# Autodesk Inventor assembly: port_starboard_side
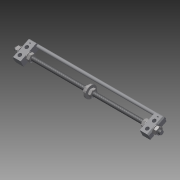
[picture p0: Inventor's stored thumbnail of the model, 180x180]
Saved by Autodesk Inventor 2015 (Build 190159000, 159)
## iProperties
Created: 2015-04-28
Part Number: port_starboard_side
Document SubType Name: Assembly
Designer: X
Author: X
## Documents named in this file (7)
- G:\3d printer\Prusa i3\CAD\port_starboard_side.iam
- G:\3d printer\Prusa i3\CAD\rod\M10-380-thread.ipt
- G:\3d printer\Prusa i3\CAD\3d_printer_part\y-corners.ipt
- G:\3d printer\Prusa i3\CAD\rod\M8-350-smooth.ipt
- D:\Inventor\Content Center Files\R2015\en-US\DIN 934\DIN 934 - M10 x 1.25.ipt
- D:\Inventor\Content Center Files\R2015\en-US\ISO 7089\ISO 7089 - 10 - 140 HV(1).ipt
- D:\Inventor\Content Center Files\R2015\en-US\ISO 7093 A\ISO 7093 A - ST 10 - 140 HV .ipt
## Components (16 placed, 6 different names)
1. M10-380-thread:1 — Cylindrical:1, Cylindrical:2, Cylindrical:3, Cylindrical:4, Cylindrical:5, Cylindrical:6, Cylindrical:7, Cylindrical:8
2. y-corners:1 — Insert:2, Cylindrical:2, Insert:5, Insert:9
3. y-corners:2 — Insert:3, Cylindrical:1, Insert:4, Insert:8
4. M8-350-smooth:1 — Insert:2, Insert:3
5. ISO 7089 10 - 140 HV:2 — Insert:5, Insert:7
6. ISO 7089 10 - 140 HV:1 — Insert:4, Insert:6
7. DIN 934 - replaced by DIN EN 24032/28673/28674 M10 x 1.25:1 — Insert:7
8. DIN 934 - replaced by DIN EN 24032/28673/28674 M10 x 1.25:2 — Insert:6
9. ISO 7089 10 - 140 HV:3 — Insert:8, Mate:1
10. ISO 7089 10 - 140 HV:4 — Insert:9, Mate:2
11. DIN 934 - replaced by DIN EN 24032/28673/28674 M10 x 1.25:3 — Cylindrical:3, Mate:1
12. DIN 934 - replaced by DIN EN 24032/28673/28674 M10 x 1.25:4 — Cylindrical:4, Mate:2
13. ISO 7093 A ST 10 - 140 HV - A:1 — Cylindrical:5, Mate:3, Mate:4
14. ISO 7093 A ST 10 - 140 HV - A:2 — Cylindrical:6, Mate:3, Mate:5
15. DIN 934 - replaced by DIN EN 24032/28673/28674 M10 x 1.25:5 — Cylindrical:8, Mate:4
16. DIN 934 - replaced by DIN EN 24032/28673/28674 M10 x 1.25:6 — Cylindrical:7, Mate:5
## Relationships (21: Insert 8, CylindricalJoint 8, Mate 5)
- Insert:2: y-corners:1 ↔ M8-350-smooth:1
- Insert:3: y-corners:2 ↔ M8-350-smooth:1
- Cylindrical:1: M10-380-thread:1 ↔ y-corners:2
- Cylindrical:2: M10-380-thread:1 ↔ y-corners:1
- Insert:4: y-corners:2 ↔ ISO 7089 10 - 140 HV:1
- Insert:5: y-corners:1 ↔ ISO 7089 10 - 140 HV:2
- Insert:6: ISO 7089 10 - 140 HV:1 ↔ DIN 934 - replaced by DIN EN 24032/28673/28674 M10 x 1.25:2
- Insert:7: ISO 7089 10 - 140 HV:2 ↔ DIN 934 - replaced by DIN EN 24032/28673/28674 M10 x 1.25:1
- Insert:8: y-corners:2 ↔ ISO 7089 10 - 140 HV:3
- Insert:9: y-corners:1 ↔ ISO 7089 10 - 140 HV:4
- Cylindrical:3: M10-380-thread:1 ↔ DIN 934 - replaced by DIN EN 24032/28673/28674 M10 x 1.25:3
- Mate:1: ISO 7089 10 - 140 HV:3 ↔ DIN 934 - replaced by DIN EN 24032/28673/28674 M10 x 1.25:3
- Cylindrical:4: M10-380-thread:1 ↔ DIN 934 - replaced by DIN EN 24032/28673/28674 M10 x 1.25:4
- Mate:2: ISO 7089 10 - 140 HV:4 ↔ DIN 934 - replaced by DIN EN 24032/28673/28674 M10 x 1.25:4
- Cylindrical:5: M10-380-thread:1 ↔ ISO 7093 A ST 10 - 140 HV - A:1
- Cylindrical:6: M10-380-thread:1 ↔ ISO 7093 A ST 10 - 140 HV - A:2
- Cylindrical:7: M10-380-thread:1 ↔ DIN 934 - replaced by DIN EN 24032/28673/28674 M10 x 1.25:6
- Cylindrical:8: M10-380-thread:1 ↔ DIN 934 - replaced by DIN EN 24032/28673/28674 M10 x 1.25:5
- Mate:3: ISO 7093 A ST 10 - 140 HV - A:1 ↔ ISO 7093 A ST 10 - 140 HV - A:2
- Mate:4: ISO 7093 A ST 10 - 140 HV - A:1 ↔ DIN 934 - replaced by DIN EN 24032/28673/28674 M10 x 1.25:5
- Mate:5: ISO 7093 A ST 10 - 140 HV - A:2 ↔ DIN 934 - replaced by DIN EN 24032/28673/28674 M10 x 1.25:6
